# Autodesk Inventor assembly: Skrzydło
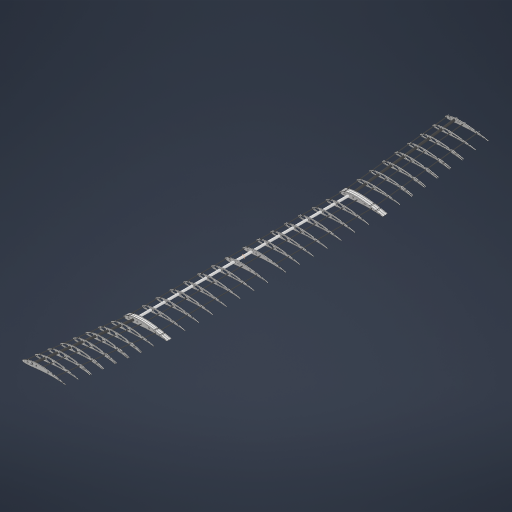
[picture p0: Inventor's stored thumbnail of the model, 512x512]
Saved by Autodesk Inventor 2023 (Build 270158000, 158)
## iProperties
Created: 2023-01-05
Part Number: Skrzydło
Document SubType Name: Assembly
Designer: szykr
Author: szykr
## Documents named in this file (8)
- D:\Folder Instalacyjny\GitHub Pliki\Solaris\new model\Skrzydło.iam
- D:\Folder Instalacyjny\GitHub Pliki\Solaris\new model\wingspar.ipt
- D:\Folder Instalacyjny\GitHub Pliki\Solaris\new model\Żerbo montaż.ipt
- D:\Folder Instalacyjny\GitHub Pliki\Solaris\new model\Żebro default.ipt
- D:\Folder Instalacyjny\GitHub Pliki\Solaris\new model\kuplung.ipt
- D:\Folder Instalacyjny\GitHub Pliki\Solaris\new model\skrzydlo_ster.iam
- D:\Folder Instalacyjny\GitHub Pliki\Solaris\new model\cienki_spar_dlugi.ipt
- D:\Folder Instalacyjny\GitHub Pliki\Solaris\new model\cienki_spar_krotki.ipt
## Components (25 placed, 7 different names)
1. wingspar:1 — Insert:1, Insert:2
2. Żerbo montaż:1 — Insert:1, Insert:3, Insert:4, Insert:14
3. Żerbo montaż:2 — Insert:2, Insert:5, Insert:6, Insert:13
4. Żerbo montaż:3 — Insert:4, Insert:7
5. Żerbo montaż:4 — Insert:6, Insert:8, Insert:11
6. kuplung:1 — Insert:7, Insert:9
7. kuplung:2 — Insert:8, Insert:12, Insert:15
8. skrzydlo_ster:1 [sub-assembly] — Insert:9
9. skrzydlo_ster:2 [sub-assembly] — Insert:15
10. cienki_spar_dlugi:1 — Insert:11
11. cienki_spar_dlugi:2 — Insert:12
12. cienki_spar_krotki:1 — Insert:13
13. cienki_spar_krotki:2 — Insert:14
14. Żebro default:1 — Insert:3
15. Żebro default:2
16. Żebro default:3
17. Żebro default:4
18. Żebro default:5
19. Żebro default:6
20. Żebro default:7 — Insert:5
21. Żebro default:8
22. Żebro default:9
23. Żebro default:10
24. Żebro default:11
25. Żebro default:12
## Component patterns: (6 elements, first: Żebro default:1), (6 elements, first: Żebro default:7)
## Relationships (14: Insert 14)
- Insert:1 (-460 mm): wingspar:1 ↔ Żerbo montaż:1
- Insert:2 (-460 mm): wingspar:1 ↔ Żerbo montaż:2
- Insert:3 (-64.1429 mm): Żerbo montaż:1 ↔ Żebro default:1
- Insert:4 (449 mm): Żerbo montaż:1 ↔ Żerbo montaż:3
- Insert:5 (-64.1429 mm): Żerbo montaż:2 ↔ Żebro default:7
- Insert:6 (449 mm): Żerbo montaż:2 ↔ Żerbo montaż:4
- Insert:7: Żerbo montaż:3 ↔ kuplung:1
- Insert:8: Żerbo montaż:4 ↔ kuplung:2
- Insert:9: kuplung:1 ↔ skrzydlo_ster:1
- Insert:11 (-8.968 mm): Żerbo montaż:4 ↔ cienki_spar_dlugi:1
- Insert:12 (-8.448 mm): kuplung:2 ↔ cienki_spar_dlugi:2
- Insert:13: Żerbo montaż:2 ↔ cienki_spar_krotki:1
- Insert:14: Żerbo montaż:1 ↔ cienki_spar_krotki:2
- Insert:15: kuplung:2 ↔ skrzydlo_ster:2
## Named parameters: ilosc_cala_zeber = 8, ilosc_zeber_pattern = 6, dlugosc_zeber = 449 mm, spacing = 64.14286 mm
